# Autodesk Inventor assembly: RT_FRM_A_Left_Front_Cover_MIR
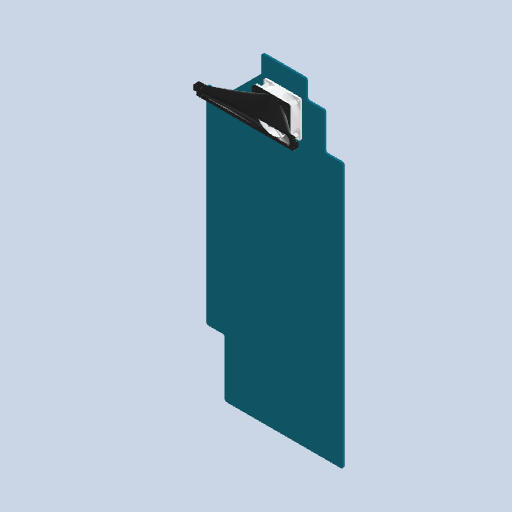
[picture p0: Inventor's stored thumbnail of the model, 512x512]
Saved by Autodesk Inventor 2025.3 (Build 293356000, 356)
## iProperties
Created: 2026-06-07
Part Number: RT_FRM_A_Left_Front_Cover_MIR
Document SubType Name: Assembly
Designer: louis
Author: louis
## Documents named in this file (4)
- C:\Users\louis\OneDrive\Desktop\R_Trident\02_CAD\04_Subassemblies\TEMP_MIR_Front_Cover\RT_FRM_A_Left_Front_Cover_MIR.iam
- C:\Users\louis\OneDrive\Desktop\R_Trident\02_CAD\04_Subassemblies\TEMP_MIR_Front_Cover\RT_FRM_MC_014_FrontCover_L_MIR.ipt
- C:\Users\louis\OneDrive\Desktop\R_Trident\02_CAD\04_Subassemblies\TEMP_MIR_Front_Cover\RT_ELE_PR_015_AirDuct_MIR.ipt
- C:\Users\louis\OneDrive\Desktop\R_Trident\02_CAD\04_Subassemblies\TEMP_MIR_Front_Cover\NF-R8_Public-CAD_MIR.iam
## Components (3 placed, 3 different names)
1. RT_FRM_MC_014_FrontCover_L_MIR:1 — Mate:2, Mate:1, Mate:5, Mate:4, Mate:3
2. RT_ELE_PR_015_AirDuct_MIR:1 — Mate:7, Mate:6
3. NF-R8_Public-CAD_MIR:1 [sub-assembly] — Mate:7, Mate:6, Mate:5, Mate:4, Mate:3
## Relationships (7: Mate 7)
- Mate:2: RT_FRM_MC_014_FrontCover_L_MIR:1
- Mate:1: RT_FRM_MC_014_FrontCover_L_MIR:1
- Mate:7: RT_ELE_PR_015_AirDuct_MIR:1 ↔ NF-R8_Public-CAD_MIR:1
- Mate:6: RT_ELE_PR_015_AirDuct_MIR:1 ↔ NF-R8_Public-CAD_MIR:1
- Mate:5: RT_FRM_MC_014_FrontCover_L_MIR:1 ↔ NF-R8_Public-CAD_MIR:1
- Mate:4: RT_FRM_MC_014_FrontCover_L_MIR:1 ↔ NF-R8_Public-CAD_MIR:1
- Mate:3: RT_FRM_MC_014_FrontCover_L_MIR:1 ↔ NF-R8_Public-CAD_MIR:1
